# Autodesk Inventor assembly: wheel_dual_MIR
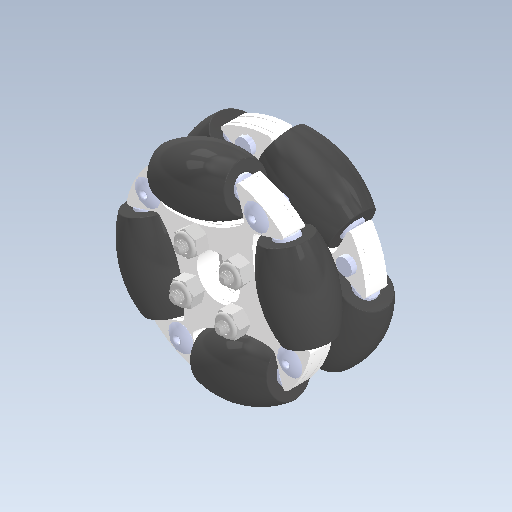
[picture p0: Inventor's stored thumbnail of the model, 512x512]
Saved by Autodesk Inventor 2020 (Build 240168000, 168)
## iProperties
Created: 2019-11-04
Part Number: wheel_dual_MIR
Document SubType Name: Assembly
Designer: jackm
Author: ball
## Documents named in this file (5)
- D:\FTC8863\2019 Robot\Odoemetry module\wheel_dual_MIR.iam
- D:\FTC8863\2019 Robot\Odoemetry module\wheel single_MIR.iam
- D:\FTC8863\2019 Robot\Odoemetry module\Our omiwheelinsert_MIR.ipt
- D:\FTC8863\2019 Robot\Odoemetry module\91292A031_TYPE 18-8 SS SOCKET HEAD CAP SCREW_MIR.ipt
- D:\FTC8863\2019 Robot\Odoemetry module\93625A101_TYPE 18-8 M2 STAINLESS STL NYLON-INSERT LOCKNUT_MIR.ipt
## Components (11 placed, 4 different names)
1. wheel single_MIR:1 [sub-assembly] — Mate:5, Mate:2, Mate:1, Mate:10, Mate:9, Mate:18, Mate:17, Mate:16, Mate:8, Mate:7
2. wheel single_MIR:2 [sub-assembly] — Mate:5, Mate:6, Mate:4, Mate:15, Mate:12, Mate:22, Mate:21, Mate:14
3. Our omiwheelinsert_MIR:1 — Mate:6, Mate:4, Mate:2, Mate:1
4. 91292A031_TYPE 18-8 SS SOCKET HEAD CAP SCREW_MIR:1 — Mate:10, Mate:9, Mate:13
5. 91292A031_TYPE 18-8 SS SOCKET HEAD CAP SCREW_MIR:2 — Mate:18, Mate:17, Mate:20
6. 91292A031_TYPE 18-8 SS SOCKET HEAD CAP SCREW_MIR:3 — Mate:16, Mate:15, Mate:19
7. 91292A031_TYPE 18-8 SS SOCKET HEAD CAP SCREW_MIR:4 — Mate:8, Mate:7, Mate:11
8. 93625A101_TYPE 18-8 M2 STAINLESS STL NYLON-INSERT LOCKNUT_MIR:1 — Mate:12, Mate:11
9. 93625A101_TYPE 18-8 M2 STAINLESS STL NYLON-INSERT LOCKNUT_MIR:2 — Mate:22, Mate:20
10. 93625A101_TYPE 18-8 M2 STAINLESS STL NYLON-INSERT LOCKNUT_MIR:3 — Mate:21, Mate:19
11. 93625A101_TYPE 18-8 M2 STAINLESS STL NYLON-INSERT LOCKNUT_MIR:4 — Mate:14, Mate:13
## Relationships (21: Mate 21)
- Mate:5: wheel single_MIR:1 ↔ wheel single_MIR:2
- Mate:6: wheel single_MIR:2 ↔ Our omiwheelinsert_MIR:1
- Mate:4: wheel single_MIR:2 ↔ Our omiwheelinsert_MIR:1
- Mate:2: wheel single_MIR:1 ↔ Our omiwheelinsert_MIR:1
- Mate:1: wheel single_MIR:1 ↔ Our omiwheelinsert_MIR:1
- Mate:10: wheel single_MIR:1 ↔ 91292A031_TYPE 18-8 SS SOCKET HEAD CAP SCREW_MIR:1
- Mate:9: wheel single_MIR:1 ↔ 91292A031_TYPE 18-8 SS SOCKET HEAD CAP SCREW_MIR:1
- Mate:18: wheel single_MIR:1 ↔ 91292A031_TYPE 18-8 SS SOCKET HEAD CAP SCREW_MIR:2
- Mate:17: wheel single_MIR:1 ↔ 91292A031_TYPE 18-8 SS SOCKET HEAD CAP SCREW_MIR:2
- Mate:16: wheel single_MIR:1 ↔ 91292A031_TYPE 18-8 SS SOCKET HEAD CAP SCREW_MIR:3
- Mate:15: wheel single_MIR:2 ↔ 91292A031_TYPE 18-8 SS SOCKET HEAD CAP SCREW_MIR:3
- Mate:8: wheel single_MIR:1 ↔ 91292A031_TYPE 18-8 SS SOCKET HEAD CAP SCREW_MIR:4
- Mate:7: wheel single_MIR:1 ↔ 91292A031_TYPE 18-8 SS SOCKET HEAD CAP SCREW_MIR:4
- Mate:12: wheel single_MIR:2 ↔ 93625A101_TYPE 18-8 M2 STAINLESS STL NYLON-INSERT LOCKNUT_MIR:1
- Mate:11: 91292A031_TYPE 18-8 SS SOCKET HEAD CAP SCREW_MIR:4 ↔ 93625A101_TYPE 18-8 M2 STAINLESS STL NYLON-INSERT LOCKNUT_MIR:1
- Mate:22: wheel single_MIR:2 ↔ 93625A101_TYPE 18-8 M2 STAINLESS STL NYLON-INSERT LOCKNUT_MIR:2
- Mate:20: 91292A031_TYPE 18-8 SS SOCKET HEAD CAP SCREW_MIR:2 ↔ 93625A101_TYPE 18-8 M2 STAINLESS STL NYLON-INSERT LOCKNUT_MIR:2
- Mate:21: wheel single_MIR:2 ↔ 93625A101_TYPE 18-8 M2 STAINLESS STL NYLON-INSERT LOCKNUT_MIR:3
- Mate:19: 91292A031_TYPE 18-8 SS SOCKET HEAD CAP SCREW_MIR:3 ↔ 93625A101_TYPE 18-8 M2 STAINLESS STL NYLON-INSERT LOCKNUT_MIR:3
- Mate:14: wheel single_MIR:2 ↔ 93625A101_TYPE 18-8 M2 STAINLESS STL NYLON-INSERT LOCKNUT_MIR:4
- Mate:13: 91292A031_TYPE 18-8 SS SOCKET HEAD CAP SCREW_MIR:1 ↔ 93625A101_TYPE 18-8 M2 STAINLESS STL NYLON-INSERT LOCKNUT_MIR:4
